# Autodesk Inventor assembly: mizuno-pipe
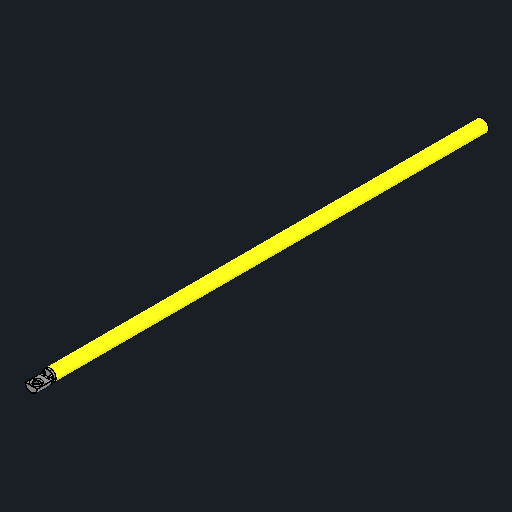
[picture p0: Inventor's stored thumbnail of the model, 512x512]
Saved by Autodesk Inventor 2027.1 (Build 311270010, 270A)
## iProperties
Created: 2026-05-08
Part Number: mizuno-pipe
Document SubType Name: Assembly
Designer: zetsu
Author: zetsu
## Documents named in this file (3)
- C:\Users\queezz\Dropbox\Drawings\pihti-cad\bellows-probe\mizuno-pipe.iam
- C:\Users\queezz\Dropbox\Drawings\pihti-cad\bellows-probe\mizuno-probe-head.iam
- C:\Users\queezz\Dropbox\Drawings\pihti-cad\bellows-probe\pipe-for-mizuno-probe.ipt
## Components (2 placed, 2 different names)
1. mizuno-probe-head:1 [sub-assembly] — Rigid:1
2. pipe-for-mizuno-probe:1 — Rigid:1
## Relationships (1: WeldJoint 1)
- Rigid:1 [WeldJoint]: mizuno-probe-head:1 ↔ pipe-for-mizuno-probe:1
